# Autodesk Inventor assembly: wimp with full update mk 2
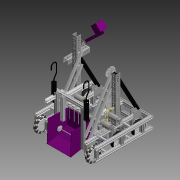
[picture p0: Inventor's stored thumbnail of the model, 180x180]
Saved by Autodesk Inventor 2013 (Build 170138000, 138)
## iProperties
Created: 2013-12-21
Part Number: wimp with full update mk 2
Document SubType Name: Assembly
Designer: kahohbein
Author: kahohbein
## Documents named in this file (38)
- C:\Users\nojessen\Documents\GitHub\2013-2014_BlockParty\CAD\wimp with full update mk 2.iam
- C:\Users\nojessen\Documents\Robotics\2013-14\CAD\Drive\Final Drive Complete\Driveopen2.iam
- C:\Users\nojessen\Documents\GitHub\2013-2014_BlockParty\CAD\COTSParts\Tetrix\Tetrix flat plate.ipt
- C:\Users\nojessen\Documents\GitHub\2013-2014_BlockParty\CAD\COTSParts\Tetrix\Tetrix channel 32mm.ipt
- C:\Users\nojessen\Documents\GitHub\2013-2014_BlockParty\CAD\COTSParts\Tetrix\Bronze bushing.ipt
- C:\Users\nojessen\Documents\GitHub\2013-2014_BlockParty\CAD\COTSParts\Tetrix\Tetrix motor mount.ipt
- C:\Users\nojessen\Documents\GitHub\2013-2014_BlockParty\CAD\Lift\MK3\hook prototype.ipt
- C:\Users\nojessen\Documents\GitHub\2013-2014_BlockParty\CAD\Lift\Bosch 20x20 modified.ipt
- C:\Users\nojessen\Documents\GitHub\2013-2014_BlockParty\CAD\four bar linkage\custom Box Aluminum.ipt
- C:\Users\nojessen\Documents\GitHub\2013-2014_BlockParty\CAD\four bar linkage\custom bosch 8in.ipt
- C:\Users\nojessen\Documents\GitHub\2013-2014_BlockParty\CAD\COTSParts\Tetrix\Tetrix Channel 416mm_CPY.ipt
- C:\Users\nojessen\Documents\GitHub\2013-2014_BlockParty\CAD\COTSParts\Tetrix\Tetrix Hub - axle.ipt
- C:\Users\nojessen\Documents\GitHub\2013-2014_BlockParty\CAD\Lift\MK4\Winch MK4.iam
- C:\Users\nojessen\Documents\GitHub\2013-2014_BlockParty\CAD\COTSParts\Fasteners\4-40 SHCS x125.ipt
- C:\Users\nojessen\Documents\GitHub\2013-2014_BlockParty\CAD\Lift\MK4\ratchet stop mk 2.ipt
- C:\Users\nojessen\Documents\GitHub\2013-2014_BlockParty\CAD\Lift\MK4\Tetrix channel 32mm modified.ipt
- C:\Users\nojessen\Documents\GitHub\2013-2014_BlockParty\CAD\Pick-up Blocks\axle.ipt
- C:\Users\nojessen\Documents\GitHub\2013-2014_BlockParty\CAD\COTSParts\Tetrix\Tetrix sprocket 16T_MIR2.ipt
- C:\Users\nojessen\Documents\GitHub\2013-2014_BlockParty\CAD\COTSParts\Tetrix\Tetrix Hub - axle_MIR2.ipt
- C:\Users\nojessen\Documents\GitHub\2013-2014_BlockParty\CAD\COTSParts\Bosch Extrusion\Gusset 20x20 w screws.ipt
- C:\Users\nojessen\Documents\GitHub\2013-2014_BlockParty\CAD\COTSParts\Tetrix\Tetrix motor mount_MIR2.ipt
- C:\Users\nojessen\Documents\GitHub\2013-2014_BlockParty\CAD\COTSParts\Tetrix\Tetrix hub - motor.ipt
- C:\Users\nojessen\Documents\GitHub\2013-2014_BlockParty\CAD\four bar linkage\Bucket.ipt
- C:\Users\nojessen\Documents\GitHub\2013-2014_BlockParty\CAD\U-Channel.ipt
- C:\Users\nojessen\Documents\GitHub\2013-2014_BlockParty\CAD\Aluminum U-Channel Holder.ipt
- C:\Users\nojessen\Documents\GitHub\2013-2014_BlockParty\CAD\COTSParts\Bosch Extrusion\Bosch 20x20.ipt
- C:\Users\nojessen\Documents\GitHub\2013-2014_BlockParty\CAD\COTSParts\Bosch Extrusion\Bosch 20x20 9 in.ipt
- C:\Users\nojessen\Documents\GitHub\2013-2014_BlockParty\CAD\COTSParts\Tetrix\Tetrix channel 160mm.ipt
- C:\Users\nojessen\Documents\GitHub\2013-2014_BlockParty\CAD\COTSParts\Tetrix\Tetrix servo 180.ipt
- C:\Users\nojessen\Documents\GitHub\2013-2014_BlockParty\CAD\COTSParts\Tetrix\Tetrix bracket - single servo.ipt
- C:\Users\nojessen\Documents\GitHub\2013-2014_BlockParty\CAD\COTSParts\Tetrix\Tetrix channel 124 mm.ipt
- C:\Users\nojessen\Documents\GitHub\2013-2014_BlockParty\CAD\COTSParts\Tetrix\Tetrix shaft 100mm_MIR2.ipt
- C:\Users\nojessen\Documents\GitHub\2013-2014_BlockParty\CAD\COTSParts\Tetrix\Tetrix motor_MIR2.ipt
- C:\Users\nojessen\Documents\GitHub\2013-2014_BlockParty\CAD\COTSParts\Tetrix\Tetrix angle 208mm.ipt
- C:\Users\nojessen\Documents\GitHub\2013-2014_BlockParty\CAD\AutoBucket.ipt
- C:\Users\nojessen\Documents\GitHub\2013-2014_BlockParty\CAD\COTSParts\Tetrix\Tetrix Gear 40T.ipt
- C:\Users\nojessen\Documents\GitHub\2013-2014_BlockParty\CAD\COTSParts\Tetrix\Tetrix Gear 80T.ipt
- C:\Users\nojessen\Documents\GitHub\2013-2014_BlockParty\CAD\COTSParts\Tetrix\Tetrix Gear 120T.ipt
## Components (77 placed, 37 different names)
1. Driveopen2:1 [sub-assembly] — Mate:1, Mate:2, Mate:3, Mate:4, Mate:5, Mate:6, Mate:230, Mate:231, Mate:232, Mate:233, Flush:22, Flush:23, Flush:24, Flush:25, Mate:236, Mate:248, Mate:250, Flush:28, Flush:29
2. Tetrix flat plate:1 — Mate:2, Mate:3, Mate:4, Mate:15, Mate:16, Mate:110, Flush:10, Mate:191, Mate:192, Mate:193
3. Tetrix flat plate:2 — Mate:1, Mate:5, Mate:6, Mate:11, Mate:12, Flush:8, Mate:176, Mate:194, Mate:195, Mate:196, Mate:199, Mate:200, Mate:229
4. Tetrix channel 32mm:1 — Mate:15, Mate:16, Flush:9, Mate:111, Flush:10
5. Tetrix channel 32mm:2 — Mate:11, Mate:12, Flush:8, Mate:228, Flush:21
6. hook prototype:1 — Mate:80, Mate:81, Angle:1
7. Bosch 20x20 modified:1 — Mate:80, Mate:81, Mate:99, Flush:6, Flush:11, Angle:1
8. custom Box Aluminum:1 — Flush:5, Mate:96, Mate:151, Mate:152, Mate:238, Mate:240
9. custom Box Aluminum:3 — Flush:5, Mate:134, Mate:155, Mate:156
10. custom Box Aluminum:4 — Flush:4, Mate:124, Mate:129, Mate:131, Mate:135, Mate:207, Mate:305, Mate:306
11. custom bosch 8in:1 — Mate:96, Mate:97, Mate:99, Flush:6, Flush:11, Flush:15, Mate:206, Mate:209, Mate:210, Mate:264, Flush:33, Mate:266
12. Tetrix Channel 416mm_CPY:1 — Mate:110, Flush:9, Mate:111, Mate:132, Mate:133, Mate:153, Mate:154, Mate:234, Mate:235, Mate:300, Mate:301, Mate:302, Mate:307, Mate:308
13. Tetrix Hub - axle:1 — Mate:124, Mate:129, Mate:131, Mate:132, Mate:133
14. custom bosch 8in:2 — Mate:134, Mate:135, Mate:137, Flush:12, Flush:13, Mate:207, Mate:208, Mate:211, Flush:16, Flush:34, Mate:267, Flush:42
15. Bosch 20x20 modified:2 — Mate:137, Flush:12, Flush:13, Mate:138, Mate:139, Angle:2
16. hook prototype:2 — Mate:138, Mate:139, Angle:2
17. Tetrix Hub - axle:2 — Mate:143, Mate:144, Mate:239, Mate:241, Mate:244, Mate:245
18. Tetrix Hub - axle:3 — Mate:151, Mate:152, Mate:238, Mate:240, Mate:242, Mate:243
19. Tetrix Hub - axle:4 — Mate:153, Mate:154, Mate:155, Mate:156
20. Winch MK4:1 [sub-assembly] — Mate:197, Mate:198, Flush:14
21. 4-40 SHCS x125:1 — Mate:179, Mate:181
22. ratchet stop mk 2:1 — Mate:177, Mate:182
23. 4-40 SHCS x125:2 — Mate:178, Mate:180
24. Tetrix channel 32mm modified:1 — Mate:176, Mate:177, Mate:178, Mate:179, Mate:180, Mate:181, Mate:182, Mate:199, Mate:200
25. ratchet stop mk 2:2 — Flush:14
26. 4-40 SHCS x125:3
27. 4-40 SHCS x125:4
28. Tetrix motor mount:1 — Mate:191, Mate:192, Mate:193, Mate:198
29. Tetrix motor mount:2 — Mate:194, Mate:195, Mate:196, Mate:197
30. Bronze bushing:13 — Mate:208, Mate:211, Mate:212, Mate:226
31. Bronze bushing:14 — Mate:209, Mate:210, Mate:217
32. axle:1 — Mate:212, Flush:16, Mate:216, Mate:227
33. Tetrix sprocket 16T_MIR2:1 — Mate:213, Mate:214, Mate:215
34. Tetrix Hub - axle_MIR2:1 — Mate:213, Mate:214, Mate:215, Mate:216, Mate:217
35. Bucket:1 — Mate:226, Mate:227
36. Tetrix Channel 416mm_CPY:2 — Mate:228, Mate:229, Flush:21, Mate:242, Mate:243, Mate:244, Mate:245, Mate:246, Mate:247, Mate:257, Mate:258
37. U-Channel:3 — Mate:234, Mate:235, Mate:237
38. Aluminum U-Channel Holder:1 — Mate:233, Flush:23, Flush:27, Mate:248
39. Aluminum U-Channel Holder:2 — Mate:231, Flush:25, Flush:26, Mate:236, Mate:237
40. Aluminum U-Channel Holder:3 — Mate:230, Flush:24, Flush:26
41. Aluminum U-Channel Holder:4 — Mate:232, Flush:22, Flush:27, Mate:249
42. U-Channel:8 — Mate:246, Mate:247, Mate:249
43. Bosch 20x20:1 — Mate:250, Flush:28, Flush:29, Mate:251, Angle:4, Mate:252, Angle:5, Mate:253, Mate:256, Angle:6
44. Gusset 20x20 w screws:3 — Mate:252, Angle:5, Mate:254, Flush:30, Angle:6
45. Gusset 20x20 w screws:4 — Mate:251, Angle:4, Mate:255, Flush:31, Flush:32
46. Bosch 20x20 9 in:1 — Mate:253, Mate:254, Flush:30, Mate:255, Flush:31, Flush:32, Mate:256
47. Tetrix channel 160mm:2 — Mate:257, Mate:258, Mate:259, Mate:260, Mate:261
48. Tetrix servo 180:2 — Mate:262, Mate:263, Mate:296, Mate:297, Mate:298
49. Tetrix bracket - single servo:2 — Mate:259, Mate:260, Mate:261, Mate:262, Mate:263
50. Bosch 20x20 9 in:3 — Mate:264, Flush:33, Flush:34, Mate:265, Flush:35, Mate:268, Mate:284, Mate:285, Flush:43, Mate:288, Mate:289
51. Bosch 20x20:2 — Mate:265, Flush:35, Mate:266, Flush:44
52. Tetrix channel 124 mm:1 — Mate:267, Mate:268, Flush:37, Mate:270, Mate:274, Mate:275, Mate:276, Mate:277, Mate:278, Mate:279, Mate:284, Flush:42
53. Tetrix Hub - axle_MIR2:2 — Mate:269, Flush:36, Flush:37
54. Tetrix Hub - axle_MIR2:3 — Mate:271, Flush:38, Mate:276
55. Tetrix Hub - axle_MIR2:4 — Mate:272, Flush:39, Mate:274
56. Tetrix Hub - axle_MIR2:5 — Mate:273, Flush:40, Mate:278
57. Tetrix shaft 100mm_MIR2:1 — Mate:269, Flush:36, Mate:270
58. Tetrix shaft 100mm_MIR2:2 — Mate:273, Flush:40, Mate:279
59. Tetrix shaft 100mm_MIR2:3 — Mate:271, Flush:38, Mate:277
60. Tetrix shaft 100mm_MIR2:4 — Mate:272, Flush:39, Mate:275
61. Bosch 20x20 modified:4 — Mate:285, Flush:43, Flush:44, Mate:286, Mate:287, Mate:290, Flush:45, Mate:291, Flush:46, Flush:47
62. Bosch 20x20 modified:5
63. Gusset 20x20 w screws:5 — Mate:289, Mate:290, Flush:45
64. Gusset 20x20 w screws:6 — Mate:286, Mate:287, Mate:288
65. Tetrix motor mount_MIR2:2 — Mate:291, Flush:46, Flush:47, Mate:292, Flush:48
66. Tetrix motor_MIR2:2 — Mate:292, Flush:48, Mate:293, Mate:294
67. Tetrix sprocket 16T_MIR2:2 — Mate:293, Mate:295
68. Tetrix hub - motor:1 — Mate:294, Mate:295
69. Tetrix angle 208mm:1 — Mate:296, Mate:297, Mate:298, Mate:299, Flush:49, Flush:50
70. AutoBucket:1 — Mate:299, Flush:49, Flush:50
71. Tetrix motor_MIR2:3 — Mate:303, Flush:51, Mate:304
72. Tetrix motor mount_MIR2:3 — Mate:300, Mate:301, Mate:302, Mate:303, Flush:51
73. Tetrix Gear 40T:1 — Mate:309, Mate:310
74. Tetrix Gear 80T:1 — Mate:305, Mate:306
75. Tetrix Gear 120T:1 — Mate:307, Mate:308, Mate:309, Mate:310
76. Tetrix Gear 40T:2 — Mate:304
77. custom Box Aluminum:2 — Flush:4, Mate:97, Mate:143, Mate:144, Mate:206, Mate:239, Mate:241
## Relationships (192: Mate 145, Flush 42, Angle 5)
- Mate:1: Driveopen2:1 ↔ Tetrix flat plate:2
- Mate:2: Driveopen2:1 ↔ Tetrix flat plate:1
- Mate:3 (139.7 mm): Driveopen2:1 ↔ Tetrix flat plate:1
- Mate:4 (63.5 mm): Driveopen2:1 ↔ Tetrix flat plate:1
- Mate:5 (139.7 mm): Driveopen2:1 ↔ Tetrix flat plate:2
- Mate:6 (63.5 mm): Driveopen2:1 ↔ Tetrix flat plate:2
- Mate:11: Tetrix flat plate:2 ↔ Tetrix channel 32mm:2
- Mate:12: Tetrix flat plate:2 ↔ Tetrix channel 32mm:2
- Mate:15: Tetrix flat plate:1 ↔ Tetrix channel 32mm:1
- Mate:16: Tetrix flat plate:1 ↔ Tetrix channel 32mm:1
- Mate:80: hook prototype:1 ↔ Bosch 20x20 modified:1
- Mate:81: hook prototype:1 ↔ Bosch 20x20 modified:1
- Flush:4: custom Box Aluminum:4 ↔ custom Box Aluminum:2
- Flush:5: custom Box Aluminum:1 ↔ custom Box Aluminum:3
- Mate:96: custom Box Aluminum:1 ↔ custom bosch 8in:1
- Mate:97: custom bosch 8in:1 ↔ custom Box Aluminum:2
- Mate:99: Bosch 20x20 modified:1 ↔ custom bosch 8in:1
- Flush:6: Bosch 20x20 modified:1 ↔ custom bosch 8in:1
- Flush:8: Tetrix flat plate:2 ↔ Tetrix channel 32mm:2
- Mate:110: Tetrix flat plate:1 ↔ Tetrix Channel 416mm_CPY:1
- Flush:9: Tetrix channel 32mm:1 ↔ Tetrix Channel 416mm_CPY:1
- Mate:111: Tetrix channel 32mm:1 ↔ Tetrix Channel 416mm_CPY:1
- Flush:10: Tetrix flat plate:1 ↔ Tetrix channel 32mm:1
- Flush:11 (60.833 mm): Bosch 20x20 modified:1 ↔ custom bosch 8in:1
- Mate:124: custom Box Aluminum:4 ↔ Tetrix Hub - axle:1
- Mate:129: custom Box Aluminum:4 ↔ Tetrix Hub - axle:1
- Mate:131: custom Box Aluminum:4 ↔ Tetrix Hub - axle:1
- Mate:132: Tetrix Channel 416mm_CPY:1 ↔ Tetrix Hub - axle:1
- Mate:133: Tetrix Channel 416mm_CPY:1 ↔ Tetrix Hub - axle:1
- Mate:134: custom Box Aluminum:3 ↔ custom bosch 8in:2
- Mate:135: custom Box Aluminum:4 ↔ custom bosch 8in:2
- Mate:137: custom bosch 8in:2 ↔ Bosch 20x20 modified:2
- Flush:12: custom bosch 8in:2 ↔ Bosch 20x20 modified:2
- Flush:13 (-60.833 mm): custom bosch 8in:2 ↔ Bosch 20x20 modified:2
- Mate:138: Bosch 20x20 modified:2 ↔ hook prototype:2
- Mate:139 (-15.24 mm): Bosch 20x20 modified:2 ↔ hook prototype:2
- Mate:143: Tetrix Hub - axle:2 ↔ custom Box Aluminum:2
- Mate:144: Tetrix Hub - axle:2 ↔ custom Box Aluminum:2
- Mate:151: custom Box Aluminum:1 ↔ Tetrix Hub - axle:3
- Mate:152: custom Box Aluminum:1 ↔ Tetrix Hub - axle:3
- Mate:153: Tetrix Channel 416mm_CPY:1 ↔ Tetrix Hub - axle:4
- Mate:154: Tetrix Channel 416mm_CPY:1 ↔ Tetrix Hub - axle:4
- Mate:155: custom Box Aluminum:3 ↔ Tetrix Hub - axle:4
- Mate:156: custom Box Aluminum:3 ↔ Tetrix Hub - axle:4
- Mate:176: Tetrix flat plate:2 ↔ Tetrix channel 32mm modified:1
- Mate:177: ratchet stop mk 2:1 ↔ Tetrix channel 32mm modified:1
- Mate:178: 4-40 SHCS x125:2 ↔ Tetrix channel 32mm modified:1
- Mate:179: 4-40 SHCS x125:1 ↔ Tetrix channel 32mm modified:1
- Mate:180: 4-40 SHCS x125:2 ↔ Tetrix channel 32mm modified:1
- Mate:181: 4-40 SHCS x125:1 ↔ Tetrix channel 32mm modified:1
- Mate:182: ratchet stop mk 2:1 ↔ Tetrix channel 32mm modified:1
- Mate:191: Tetrix flat plate:1 ↔ Tetrix motor mount:1
- Mate:192: Tetrix flat plate:1 ↔ Tetrix motor mount:1
- Mate:193: Tetrix flat plate:1 ↔ Tetrix motor mount:1
- Mate:194: Tetrix flat plate:2 ↔ Tetrix motor mount:2
- Mate:195: Tetrix flat plate:2 ↔ Tetrix motor mount:2
- Mate:196: Tetrix flat plate:2 ↔ Tetrix motor mount:2
- Mate:197: Winch MK4:1 ↔ Tetrix motor mount:2
- Mate:198: Winch MK4:1 ↔ Tetrix motor mount:1
- Mate:199: Tetrix flat plate:2 ↔ Tetrix channel 32mm modified:1
- Mate:200: Tetrix flat plate:2 ↔ Tetrix channel 32mm modified:1
- Flush:14: Winch MK4:1 ↔ ratchet stop mk 2:2
- Angle:1 (90 deg): hook prototype:1 ↔ Bosch 20x20 modified:1
- Angle:2 (90 deg): Bosch 20x20 modified:2 ↔ hook prototype:2
- Flush:15 (85.9981 mm): custom bosch 8in:1
- Mate:206: custom bosch 8in:1 ↔ custom Box Aluminum:2
- Mate:207: custom Box Aluminum:4 ↔ custom bosch 8in:2
- Mate:208: custom bosch 8in:2 ↔ Bronze bushing:13
- Mate:209: custom bosch 8in:1 ↔ Bronze bushing:14
- Mate:210: custom bosch 8in:1 ↔ Bronze bushing:14
- Mate:211: custom bosch 8in:2 ↔ Bronze bushing:13
- Mate:212: Bronze bushing:13 ↔ axle:1
- Flush:16 (-17.8308 mm): custom bosch 8in:2 ↔ axle:1
- Mate:213: Tetrix sprocket 16T_MIR2:1 ↔ Tetrix Hub - axle_MIR2:1
- Mate:214: Tetrix sprocket 16T_MIR2:1 ↔ Tetrix Hub - axle_MIR2:1
- Mate:215: Tetrix sprocket 16T_MIR2:1 ↔ Tetrix Hub - axle_MIR2:1
- Mate:216: axle:1 ↔ Tetrix Hub - axle_MIR2:1
- Mate:217 (3.175 mm): Bronze bushing:14 ↔ Tetrix Hub - axle_MIR2:1
- Mate:226: Bronze bushing:13 ↔ Bucket:1
- Mate:227: axle:1 ↔ Bucket:1
- Mate:228: Tetrix channel 32mm:2 ↔ Tetrix Channel 416mm_CPY:2
- Mate:229: Tetrix flat plate:2 ↔ Tetrix Channel 416mm_CPY:2
- Flush:21: Tetrix channel 32mm:2 ↔ Tetrix Channel 416mm_CPY:2
- Mate:230: Driveopen2:1 ↔ Aluminum U-Channel Holder:3
- Mate:231: Driveopen2:1 ↔ Aluminum U-Channel Holder:2
- Mate:232: Driveopen2:1 ↔ Aluminum U-Channel Holder:4
- Mate:233: Driveopen2:1 ↔ Aluminum U-Channel Holder:1
- Flush:22: Driveopen2:1 ↔ Aluminum U-Channel Holder:4
- Flush:23: Driveopen2:1 ↔ Aluminum U-Channel Holder:1
- Flush:24: Driveopen2:1 ↔ Aluminum U-Channel Holder:3
- Flush:25: Driveopen2:1 ↔ Aluminum U-Channel Holder:2
- Mate:234: Tetrix Channel 416mm_CPY:1 ↔ U-Channel:3
- Mate:235 (1.778 mm): Tetrix Channel 416mm_CPY:1 ↔ U-Channel:3
- Flush:26: Aluminum U-Channel Holder:2 ↔ Aluminum U-Channel Holder:3
- Mate:236: Driveopen2:1 ↔ Aluminum U-Channel Holder:2
- Mate:237: U-Channel:3 ↔ Aluminum U-Channel Holder:2
- Mate:238: custom Box Aluminum:1 ↔ Tetrix Hub - axle:3
- Mate:239: Tetrix Hub - axle:2 ↔ custom Box Aluminum:2
- Mate:240: custom Box Aluminum:1 ↔ Tetrix Hub - axle:3
- Mate:241: Tetrix Hub - axle:2 ↔ custom Box Aluminum:2
- Mate:242: Tetrix Hub - axle:3 ↔ Tetrix Channel 416mm_CPY:2
- Mate:243: Tetrix Hub - axle:3 ↔ Tetrix Channel 416mm_CPY:2
- Mate:244: Tetrix Hub - axle:2 ↔ Tetrix Channel 416mm_CPY:2
- Mate:245: Tetrix Hub - axle:2 ↔ Tetrix Channel 416mm_CPY:2
- Mate:246: Tetrix Channel 416mm_CPY:2 ↔ U-Channel:8
- Mate:247 (1.778 mm): Tetrix Channel 416mm_CPY:2 ↔ U-Channel:8
- Flush:27: Aluminum U-Channel Holder:1 ↔ Aluminum U-Channel Holder:4
- Mate:248: Driveopen2:1 ↔ Aluminum U-Channel Holder:1
- Mate:249: Aluminum U-Channel Holder:4 ↔ U-Channel:8
- Mate:250: Driveopen2:1 ↔ Bosch 20x20:1
- Flush:28: Driveopen2:1 ↔ Bosch 20x20:1
- Flush:29 (-12.7 mm): Driveopen2:1 ↔ Bosch 20x20:1
- Mate:251: Bosch 20x20:1 ↔ Gusset 20x20 w screws:4
- Angle:4 (45 deg): Bosch 20x20:1 ↔ Gusset 20x20 w screws:4
- Mate:252: Bosch 20x20:1 ↔ Gusset 20x20 w screws:3
- Angle:5 (-45 deg): Bosch 20x20:1 ↔ Gusset 20x20 w screws:3
- Mate:253: Bosch 20x20:1 ↔ Bosch 20x20 9 in:1
- Mate:254: Gusset 20x20 w screws:3 ↔ Bosch 20x20 9 in:1
- Flush:30: Gusset 20x20 w screws:3 ↔ Bosch 20x20 9 in:1
- Mate:255: Gusset 20x20 w screws:4 ↔ Bosch 20x20 9 in:1
- Flush:31: Gusset 20x20 w screws:4 ↔ Bosch 20x20 9 in:1
- Flush:32: Gusset 20x20 w screws:4 ↔ Bosch 20x20 9 in:1
- Mate:256: Bosch 20x20:1 ↔ Bosch 20x20 9 in:1
- Angle:6 (-45 deg): Bosch 20x20:1 ↔ Gusset 20x20 w screws:3
- Mate:257: Tetrix Channel 416mm_CPY:2 ↔ Tetrix channel 160mm:2
- Mate:258: Tetrix Channel 416mm_CPY:2 ↔ Tetrix channel 160mm:2
- Mate:259: Tetrix channel 160mm:2 ↔ Tetrix bracket - single servo:2
- Mate:260: Tetrix channel 160mm:2 ↔ Tetrix bracket - single servo:2
- Mate:261: Tetrix channel 160mm:2 ↔ Tetrix bracket - single servo:2
- Mate:262: Tetrix servo 180:2 ↔ Tetrix bracket - single servo:2
- Mate:263: Tetrix servo 180:2 ↔ Tetrix bracket - single servo:2
- Mate:264: custom bosch 8in:1 ↔ Bosch 20x20 9 in:3
- Flush:33: custom bosch 8in:1 ↔ Bosch 20x20 9 in:3
- Flush:34: custom bosch 8in:2 ↔ Bosch 20x20 9 in:3
- Mate:265: Bosch 20x20 9 in:3 ↔ Bosch 20x20:2
- Flush:35: Bosch 20x20 9 in:3 ↔ Bosch 20x20:2
- Mate:266 (22.86 mm): custom bosch 8in:1 ↔ Bosch 20x20:2
- Mate:267 (2.54 mm): custom bosch 8in:2 ↔ Tetrix channel 124 mm:1
- Mate:268: Bosch 20x20 9 in:3 ↔ Tetrix channel 124 mm:1
- Mate:269: Tetrix Hub - axle_MIR2:2 ↔ Tetrix shaft 100mm_MIR2:1
- Flush:36: Tetrix Hub - axle_MIR2:2 ↔ Tetrix shaft 100mm_MIR2:1
- Flush:37 (2.54 mm): Tetrix channel 124 mm:1 ↔ Tetrix Hub - axle_MIR2:2
- Mate:270: Tetrix channel 124 mm:1 ↔ Tetrix shaft 100mm_MIR2:1
- Mate:271: Tetrix Hub - axle_MIR2:3 ↔ Tetrix shaft 100mm_MIR2:3
- Flush:38: Tetrix Hub - axle_MIR2:3 ↔ Tetrix shaft 100mm_MIR2:3
- Mate:272: Tetrix Hub - axle_MIR2:4 ↔ Tetrix shaft 100mm_MIR2:4
- Flush:39: Tetrix Hub - axle_MIR2:4 ↔ Tetrix shaft 100mm_MIR2:4
- Mate:273: Tetrix Hub - axle_MIR2:5 ↔ Tetrix shaft 100mm_MIR2:2
- Flush:40: Tetrix Hub - axle_MIR2:5 ↔ Tetrix shaft 100mm_MIR2:2
- Mate:274 (-9.144 mm): Tetrix channel 124 mm:1 ↔ Tetrix Hub - axle_MIR2:4
- Mate:275: Tetrix channel 124 mm:1 ↔ Tetrix shaft 100mm_MIR2:4
- Mate:276 (-9.144 mm): Tetrix channel 124 mm:1 ↔ Tetrix Hub - axle_MIR2:3
- Mate:277: Tetrix channel 124 mm:1 ↔ Tetrix shaft 100mm_MIR2:3
- Mate:278 (-9.144 mm): Tetrix channel 124 mm:1 ↔ Tetrix Hub - axle_MIR2:5
- Mate:279: Tetrix channel 124 mm:1 ↔ Tetrix shaft 100mm_MIR2:2
- Mate:284: Bosch 20x20 9 in:3 ↔ Tetrix channel 124 mm:1
- Flush:42 (-31.75 mm): custom bosch 8in:2 ↔ Tetrix channel 124 mm:1
- Mate:285: Bosch 20x20 9 in:3 ↔ Bosch 20x20 modified:4
- Flush:43: Bosch 20x20 9 in:3 ↔ Bosch 20x20 modified:4
- Flush:44: Bosch 20x20:2 ↔ Bosch 20x20 modified:4
- Mate:286: Bosch 20x20 modified:4 ↔ Gusset 20x20 w screws:6
- Mate:287: Bosch 20x20 modified:4 ↔ Gusset 20x20 w screws:6
- Mate:288: Bosch 20x20 9 in:3 ↔ Gusset 20x20 w screws:6
- Mate:289: Bosch 20x20 9 in:3 ↔ Gusset 20x20 w screws:5
- Mate:290: Bosch 20x20 modified:4 ↔ Gusset 20x20 w screws:5
- Flush:45: Bosch 20x20 modified:4 ↔ Gusset 20x20 w screws:5
- Mate:291: Bosch 20x20 modified:4 ↔ Tetrix motor mount_MIR2:2
- Flush:46 (31.75 mm): Bosch 20x20 modified:4 ↔ Tetrix motor mount_MIR2:2
- Flush:47: Bosch 20x20 modified:4 ↔ Tetrix motor mount_MIR2:2
- Mate:292: Tetrix motor mount_MIR2:2 ↔ Tetrix motor_MIR2:2
- Flush:48: Tetrix motor mount_MIR2:2 ↔ Tetrix motor_MIR2:2
- Mate:293: Tetrix motor_MIR2:2 ↔ Tetrix sprocket 16T_MIR2:2
- Mate:294: Tetrix motor_MIR2:2 ↔ Tetrix hub - motor:1
- Mate:295: Tetrix sprocket 16T_MIR2:2 ↔ Tetrix hub - motor:1
- Mate:296: Tetrix servo 180:2 ↔ Tetrix angle 208mm:1
- Mate:297: Tetrix servo 180:2 ↔ Tetrix angle 208mm:1
- Mate:298: Tetrix servo 180:2 ↔ Tetrix angle 208mm:1
- Mate:299: Tetrix angle 208mm:1 ↔ AutoBucket:1
- Flush:49: Tetrix angle 208mm:1 ↔ AutoBucket:1
- Flush:50 (-19.05 mm): Tetrix angle 208mm:1 ↔ AutoBucket:1
- Mate:300: Tetrix Channel 416mm_CPY:1 ↔ Tetrix motor mount_MIR2:3
- Mate:301: Tetrix Channel 416mm_CPY:1 ↔ Tetrix motor mount_MIR2:3
- Mate:302: Tetrix Channel 416mm_CPY:1 ↔ Tetrix motor mount_MIR2:3
- Mate:303: Tetrix motor_MIR2:3 ↔ Tetrix motor mount_MIR2:3
- Flush:51: Tetrix motor_MIR2:3 ↔ Tetrix motor mount_MIR2:3
- Mate:304: Tetrix motor_MIR2:3 ↔ Tetrix Gear 40T:2
- Mate:305: custom Box Aluminum:4 ↔ Tetrix Gear 80T:1
- Mate:306: custom Box Aluminum:4 ↔ Tetrix Gear 80T:1
- Mate:307: Tetrix Channel 416mm_CPY:1 ↔ Tetrix Gear 120T:1
- Mate:308: Tetrix Channel 416mm_CPY:1 ↔ Tetrix Gear 120T:1
- Mate:309: Tetrix Gear 40T:1 ↔ Tetrix Gear 120T:1
- Mate:310: Tetrix Gear 40T:1 ↔ Tetrix Gear 120T:1
